# Autodesk Inventor assembly: cross support
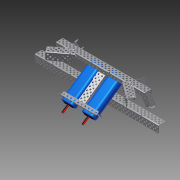
[picture p0: Inventor's stored thumbnail of the model, 180x180]
Saved by Autodesk Inventor 2014 SP1 (Build 180222100, 222)
## iProperties
Created: 2013-10-20
Part Number: cross support
Document SubType Name: Assembly
Designer: RyanHughes
Author: RyanHughes
## Documents named in this file (14)
- C:\Users\Ryan\Desktop\sw\toss up 2ed A bot\drivetrain\cross support\cross support.iam
- C:\Users\Ryan\Desktop\sw\lib\Aperture VEX CAD Library\Metal\C Channel\2 x 25.ipt
- C:\Users\Ryan\Desktop\sw\lib\Aperture VEX CAD Library\Metal\C Channel\2 x 6.ipt
- C:\Users\Ryan\Desktop\sw\lib\Aperture VEX CAD Library\Hardware\8-32\8-32_.375.ipt
- C:\Users\Ryan\Desktop\sw\lib\Aperture VEX CAD Library\Metal\L Bar\2 x 6.ipt
- C:\Users\Ryan\Desktop\sw\lib\Aperture VEX CAD Library\Hardware\8-32\8-32_.500.ipt
- C:\Users\Ryan\Desktop\sw\lib\Aperture VEX CAD Library\Spacers\SPACER-0500-0250.ipt
- C:\Users\Ryan\Desktop\sw\lib\Aperture VEX CAD Library\Metal\Custom 1 bar\1 x 3 bent 1bar.ipt
- C:\Users\Ryan\Desktop\sw\toss up 2ed A bot\drivetrain\cross support\2 x 3 - Bent.ipt
- C:\Users\Ryan\Desktop\sw\toss up 2ed A bot\drivetrain\cross support\1 x 5 small L.ipt
- C:\Users\Ryan\Desktop\sw\lib\Aperture VEX CAD Library\Metal\C Channel\2 x 8.ipt
- C:\Users\Ryan\Desktop\sw\lib\Aperture VEX CAD Library\Standoffs\BEAM-1000.ipt
- C:\Users\Ryan\Desktop\sw\lib\Super Sonic Sparks VEX CAD Library\Other Parts\7.2V (Robot Battery) NiMH 3000mAh.ipt
- C:\Users\Ryan\Desktop\sw\lib\Aperture VEX CAD Library\Metal\L Bar\2 x 35.ipt
## Components (31 placed, 12 different names)
1. 2 x 25:1 — Mate:1, Mate:2, Mate:3, Mate:4, Mate:7, Mate:11, Mate:12, Mate:16, Flush:1, Flush:2, Mate:31, Mate:40, Mate:41, Mate:42, Mate:43, Mate:44, Mate:45, Mate:48, Mate:49, Flush:9, Angle:1, Angle:2
2. 2 x 6:1 — Mate:1, Mate:5, Mate:6, Mate:17, Mate:18, Mate:19, Mate:20, Mate:21, Mate:22, Mate:23, Mate:26, Angle:1
3. 8-32_.375:1 — Mate:2, Mate:3, Mate:4, Mate:5, Mate:6
4. 2 x 6:2 — Mate:7, Mate:8, Mate:9, Mate:10, Mate:13, Mate:14, Mate:15
5. 8-32_.375:2 — Mate:8, Mate:9, Mate:10, Mate:11, Mate:12
6. 8-32_.375:3 — Mate:13, Mate:14, Mate:15, Mate:16
7. 8-32_.500:1 — Mate:17, Mate:21, Mate:22, Mate:24, Mate:30
8. 8-32_.500:2 — Mate:18, Mate:19, Mate:20, Mate:25
9. SPACER-0500-0250:1 — Mate:23, Mate:24, Mate:27
10. SPACER-0500-0250:2 — Mate:25, Mate:26, Mate:28, Mate:29
11. 1 x 3 bent 1bar:1 — Mate:27, Mate:28, Mate:29, Mate:30, Flush:12, Mate:72, Mate:73
12. 2 x 3 - Bent:1 — Flush:1, Flush:2, Flush:3, Flush:4, Mate:31, Mate:32
13. 2 x 8:1 — Flush:3, Flush:4, Mate:32, Mate:33, Flush:7, Flush:8, Tangent:1, Tangent:2
14. 1 x 5 small L:1 — Mate:33, Flush:7, Flush:8, Mate:34, Mate:35, Mate:36, Mate:37, Mate:38, Mate:39, Mate:46, Mate:47
15. BEAM-1000:1 — Mate:34, Mate:35, Mate:36
16. BEAM-1000:2 — Mate:37, Mate:38, Mate:39
17. BEAM-1000:3 — Mate:40, Mate:41, Mate:42
18. BEAM-1000:4 — Mate:43, Mate:44, Mate:45
19. 7.2V (Robot Battery) NiMH 3000mAh:1 — Mate:46, Tangent:1, Mate:48
20. 7.2V (Robot Battery) NiMH 3000mAh:2 — Mate:47, Tangent:2, Mate:49
21. 2 x 6:3 — Mate:50, Mate:51, Mate:58, Mate:59, Mate:60, Mate:61, Mate:62, Mate:63, Mate:65, Mate:66
22. 8-32_.375:4 — Mate:50, Mate:51
23. 2 x 6:4 — Mate:52, Mate:53, Mate:54, Mate:55, Mate:56, Mate:57
24. 8-32_.375:5 — Mate:52, Mate:53, Mate:54
25. 8-32_.375:6 — Mate:55, Mate:56, Mate:57
26. 8-32_.500:3 — Mate:58, Mate:59, Mate:60, Mate:64, Mate:68
27. 8-32_.500:4 — Mate:61, Mate:62, Mate:63, Mate:67
28. SPACER-0500-0250:3 — Mate:64, Mate:65, Mate:71
29. SPACER-0500-0250:4 — Mate:66, Mate:67, Mate:69, Mate:70
30. 1 x 3 bent 1bar:2 — Mate:68, Mate:69, Mate:70, Mate:71
31. 2 x 35:1 — Flush:12, Angle:2, Mate:72, Mate:73
## Relationships (85: Mate 73, Flush 8, Tangent 2, Angle 2)
- Mate:1: 2 x 25:1 ↔ 2 x 6:1
- Mate:2: 2 x 25:1 ↔ 8-32_.375:1
- Mate:3 (2.3114 mm): 2 x 25:1 ↔ 8-32_.375:1
- Mate:4 (2.3114 mm): 2 x 25:1 ↔ 8-32_.375:1
- Mate:5 (2.3114 mm): 2 x 6:1 ↔ 8-32_.375:1
- Mate:6 (2.3114 mm): 2 x 6:1 ↔ 8-32_.375:1
- Mate:7: 2 x 25:1 ↔ 2 x 6:2
- Mate:8: 2 x 6:2 ↔ 8-32_.375:2
- Mate:9 (2.3114 mm): 2 x 6:2 ↔ 8-32_.375:2
- Mate:10 (2.3114 mm): 2 x 6:2 ↔ 8-32_.375:2
- Mate:11 (2.3114 mm): 2 x 25:1 ↔ 8-32_.375:2
- Mate:12 (2.3114 mm): 2 x 25:1 ↔ 8-32_.375:2
- Mate:13: 2 x 6:2 ↔ 8-32_.375:3
- Mate:14 (2.3114 mm): 2 x 6:2 ↔ 8-32_.375:3
- Mate:15 (2.3114 mm): 2 x 6:2 ↔ 8-32_.375:3
- Mate:16 (40.4114 mm): 2 x 25:1 ↔ 8-32_.375:3
- Mate:17: 2 x 6:1 ↔ 8-32_.500:1
- Mate:18: 2 x 6:1 ↔ 8-32_.500:2
- Mate:19 (2.3114 mm): 2 x 6:1 ↔ 8-32_.500:2
- Mate:20 (2.3114 mm): 2 x 6:1 ↔ 8-32_.500:2
- Mate:21 (2.3114 mm): 2 x 6:1 ↔ 8-32_.500:1
- Mate:22 (2.3114 mm): 2 x 6:1 ↔ 8-32_.500:1
- Mate:23: 2 x 6:1 ↔ SPACER-0500-0250:1
- Mate:24: 8-32_.500:1 ↔ SPACER-0500-0250:1
- Mate:25: 8-32_.500:2 ↔ SPACER-0500-0250:2
- Mate:26: 2 x 6:1 ↔ SPACER-0500-0250:2
- Mate:27: SPACER-0500-0250:1 ↔ 1 x 3 bent 1bar:1
- Mate:28 (2.3114 mm): SPACER-0500-0250:2 ↔ 1 x 3 bent 1bar:1
- Mate:29 (2.3114 mm): SPACER-0500-0250:2 ↔ 1 x 3 bent 1bar:1
- Mate:30 (2.3114 mm): 8-32_.500:1 ↔ 1 x 3 bent 1bar:1
- Flush:1: 2 x 25:1 ↔ 2 x 3 - Bent:1
- Flush:2: 2 x 25:1 ↔ 2 x 3 - Bent:1
- Flush:3: 2 x 3 - Bent:1 ↔ 2 x 8:1
- Flush:4: 2 x 3 - Bent:1 ↔ 2 x 8:1
- Mate:31: 2 x 25:1 ↔ 2 x 3 - Bent:1
- Mate:32: 2 x 3 - Bent:1 ↔ 2 x 8:1
- Mate:33: 2 x 8:1 ↔ 1 x 5 small L:1
- Flush:7: 2 x 8:1 ↔ 1 x 5 small L:1
- Flush:8: 2 x 8:1 ↔ 1 x 5 small L:1
- Mate:34: 1 x 5 small L:1 ↔ BEAM-1000:1
- Mate:35 (2.3114 mm): 1 x 5 small L:1 ↔ BEAM-1000:1
- Mate:36 (2.3114 mm): 1 x 5 small L:1 ↔ BEAM-1000:1
- Mate:37: 1 x 5 small L:1 ↔ BEAM-1000:2
- Mate:38 (2.3114 mm): 1 x 5 small L:1 ↔ BEAM-1000:2
- Mate:39 (2.3114 mm): 1 x 5 small L:1 ↔ BEAM-1000:2
- Mate:40: 2 x 25:1 ↔ BEAM-1000:3
- Mate:41 (2.3114 mm): 2 x 25:1 ↔ BEAM-1000:3
- Mate:42 (2.3114 mm): 2 x 25:1 ↔ BEAM-1000:3
- Mate:43: 2 x 25:1 ↔ BEAM-1000:4
- Mate:44 (2.3114 mm): 2 x 25:1 ↔ BEAM-1000:4
- Mate:45 (2.3114 mm): 2 x 25:1 ↔ BEAM-1000:4
- Mate:46: 1 x 5 small L:1 ↔ 7.2V (Robot Battery) NiMH 3000mAh:1
- Mate:47: 1 x 5 small L:1 ↔ 7.2V (Robot Battery) NiMH 3000mAh:2
- Tangent:1: 2 x 8:1 ↔ 7.2V (Robot Battery) NiMH 3000mAh:1
- Tangent:2: 2 x 8:1 ↔ 7.2V (Robot Battery) NiMH 3000mAh:2
- Mate:48: 2 x 25:1 ↔ 7.2V (Robot Battery) NiMH 3000mAh:1
- Mate:49: 2 x 25:1 ↔ 7.2V (Robot Battery) NiMH 3000mAh:2
- Flush:9 (-158.75 mm): 2 x 25:1
- Angle:1 (-57.06 deg): 2 x 25:1 ↔ 2 x 6:1
- Mate:50 (2.3114 mm): 2 x 6:3 ↔ 8-32_.375:4
- Mate:51 (2.3114 mm): 2 x 6:3 ↔ 8-32_.375:4
- Mate:52 (2.3114 mm): 2 x 6:4 ↔ 8-32_.375:5
- Mate:53 (2.3114 mm): 2 x 6:4 ↔ 8-32_.375:5
- Mate:54: 2 x 6:4 ↔ 8-32_.375:5
- Mate:55 (2.3114 mm): 2 x 6:4 ↔ 8-32_.375:6
- Mate:56 (2.3114 mm): 2 x 6:4 ↔ 8-32_.375:6
- Mate:57: 2 x 6:4 ↔ 8-32_.375:6
- Mate:58 (2.3114 mm): 2 x 6:3 ↔ 8-32_.500:3
- Mate:59 (2.3114 mm): 2 x 6:3 ↔ 8-32_.500:3
- Mate:60: 2 x 6:3 ↔ 8-32_.500:3
- Mate:61 (2.3114 mm): 2 x 6:3 ↔ 8-32_.500:4
- Mate:62 (2.3114 mm): 2 x 6:3 ↔ 8-32_.500:4
- Mate:63: 2 x 6:3 ↔ 8-32_.500:4
- Mate:64: 8-32_.500:3 ↔ SPACER-0500-0250:3
- Mate:65: 2 x 6:3 ↔ SPACER-0500-0250:3
- Mate:66: 2 x 6:3 ↔ SPACER-0500-0250:4
- Mate:67: 8-32_.500:4 ↔ SPACER-0500-0250:4
- Mate:68 (2.3114 mm): 8-32_.500:3 ↔ 1 x 3 bent 1bar:2
- Mate:69 (2.3114 mm): SPACER-0500-0250:4 ↔ 1 x 3 bent 1bar:2
- Mate:70 (2.3114 mm): SPACER-0500-0250:4 ↔ 1 x 3 bent 1bar:2
- Mate:71: SPACER-0500-0250:3 ↔ 1 x 3 bent 1bar:2
- Flush:12 (-25.4 mm): 1 x 3 bent 1bar:1 ↔ 2 x 35:1
- Angle:2 (0 deg): 2 x 25:1 ↔ 2 x 35:1
- Mate:72: 1 x 3 bent 1bar:1 ↔ 2 x 35:1
- Mate:73: 1 x 3 bent 1bar:1 ↔ 2 x 35:1
## Named parameters: q = 2.3114 mm
